# Autodesk Inventor assembly: 1 part 4
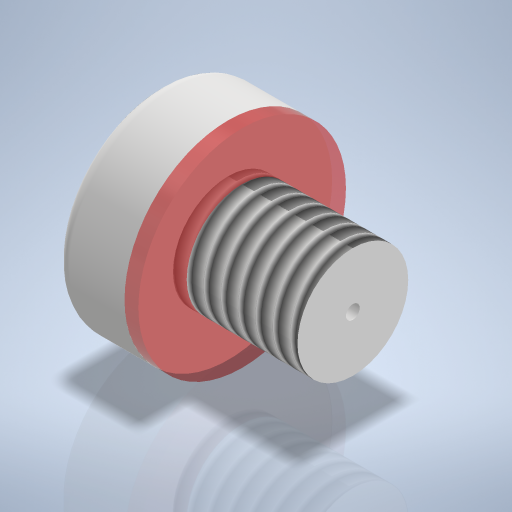
[picture p0: Inventor's stored thumbnail of the model, 512x512]
Saved by Autodesk Inventor 2024 (Build 280153000, 153)
## iProperties
Created: 2024-07-24
Part Number: 1 part 4
Document SubType Name: Assembly
Designer: ffogue
Author: ffogue
## Documents named in this file (3)
- C:\Users\ffogue\OneDrive - MuM - OM\Dokumente\Inventor\Freedom\1 part 4.iam
- C:\Users\ffogue\OneDrive - MuM - OM\Dokumente\Inventor\Freedom\1 part 4.ipt
- C:\Users\ffogue\OneDrive - MuM - OM\Dokumente\Inventor\Freedom\sicherung 1 part 4.ipt
## Components (2 placed, 2 different names)
1. 1 part 4:1 — Fluchtend:1
2. sicherung 1 part 4:1 — Fluchtend:1
## Relationships (1: Flush 1)
- Fluchtend:1 [Flush]: 1 part 4:1 ↔ sicherung 1 part 4:1
